# Autodesk Inventor assembly: Structure
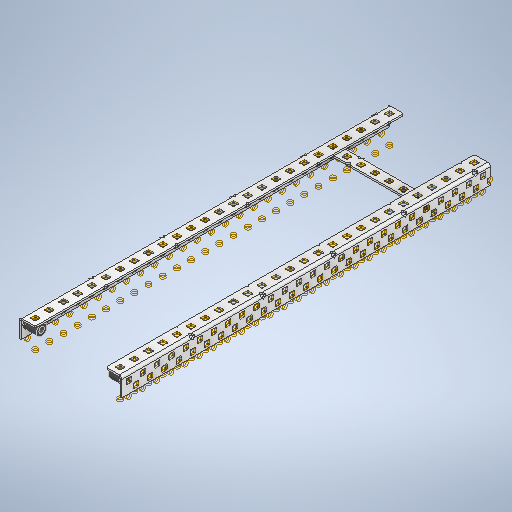
[picture p0: Inventor's stored thumbnail of the model, 512x512]
Saved by Autodesk Inventor 2025.2 (Build 292293000, 293)
## iProperties
Created: 2025-04-03
Part Number: Structure
Document SubType Name: Assembly
Designer: avere
Author: avere
## Documents named in this file (9)
- D:\vex\cad\v5\Conveyer\Structure.iam
- D:\vex\cad\VEX-CAD-Inventor\Structure\C Channel\Aluminum 1x2x1\Alu C 1x2x1x26.ipt
- D:\vex\cad\VEX-CAD-Inventor\Structure\Angle\Aluminum 1x1\Alu Angle 1x1x7.ipt
- D:\vex\cad\VEX-CAD-Inventor\Motion\Spacers\Spacer Nylon .375 OD\NSpacer .375 OD x .375.ipt
- D:\vex\cad\VEX-CAD-Inventor\Motion\Spacers\Spacer Nylon .375 OD.ipt
- D:\vex\cad\VEX-CAD-Inventor\Motion\Spacers\Washer Steel\SWasher .375 OD x .062500.ipt
- D:\vex\cad\VEX-CAD-Inventor\Motion\Spacers\Washer Steel.ipt
- D:\vex\cad\VEX-CAD-Inventor\Motion\Spacers\Washer Teflon\TWasher .375 OD x .04000.ipt
- D:\vex\cad\VEX-CAD-Inventor\Motion\Spacers\Washer Teflon.ipt
## Components (9 placed, 5 different names)
1. Alu C 1x2x1x26:1 — Flush:2, Insert:1, Insert:7
2. Alu Angle 1x1x7:1 — Mate:2, Mate:1, Insert:1, Insert:2
3. Alu C 1x2x1x26:2 — Flush:3, Insert:2, Insert:8
4. NSpacer .375 OD x .375:1 — Insert:4
5. SWasher .375 OD x .062500:1 — Insert:3, Insert:4
6. TWasher .375 OD x .04000:1 — Insert:3, Insert:8
7. NSpacer .375 OD x .375:2
8. SWasher .375 OD x .062500:2
9. TWasher .375 OD x .04000:2 — Insert:7
## Relationships (12: Insert 8, Mate 2, Flush 2)
- Mate:2 (-44.45 mm): Alu Angle 1x1x7:1
- Mate:1: Alu Angle 1x1x7:1
- Flush:2 (-165.1 mm): Alu C 1x2x1x26:1
- Insert:1: Alu C 1x2x1x26:1 ↔ Alu Angle 1x1x7:1
- Flush:3 (-165.1 mm): Alu C 1x2x1x26:2
- Insert:2: Alu Angle 1x1x7:1 ↔ Alu C 1x2x1x26:2
- Insert:3: SWasher .375 OD x .062500:1 ↔ TWasher .375 OD x .04000:1
- Insert:4: NSpacer .375 OD x .375:1 ↔ SWasher .375 OD x .062500:1
- [Insert]: SWasher .375 OD x .062500:2 ↔ TWasher .375 OD x .04000:2
- [Insert]: NSpacer .375 OD x .375:2 ↔ SWasher .375 OD x .062500:2
- Insert:7: Alu C 1x2x1x26:1 ↔ TWasher .375 OD x .04000:2
- Insert:8: Alu C 1x2x1x26:2 ↔ TWasher .375 OD x .04000:1
## Named parameters: d10_d8 = 0 mm, d11_d9 = 0 mm
